# Autodesk Inventor assembly: Z Axis FR
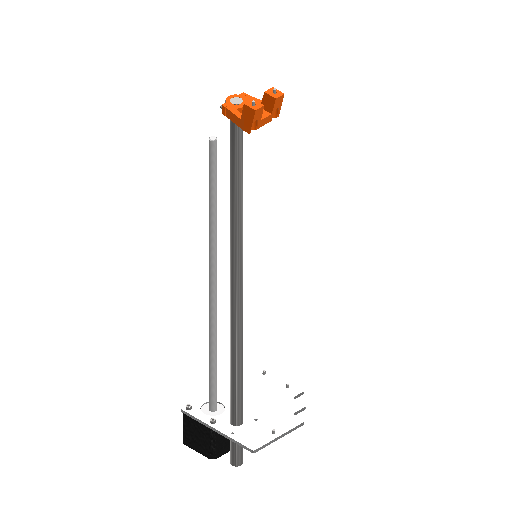
[picture p0: Inventor's stored thumbnail of the model, 512x512]
Saved by Autodesk Inventor 2023.2 (Build 272271000, 271)
## iProperties
Created: 2023-02-02
Part Number: Z Axis FR
Document SubType Name: Assembly
Designer: remop
Author: remop
## Documents named in this file (9)
- C:\Users\remop\OneDrive\Documents\Inventor\3D Printers\LuEVO\Mk5_FullKinematic\Z Axis Front Right.iam
- C:\Users\remop\OneDrive\Documents\Inventor\3D Printers\LuEVO\Mk5_FullKinematic\Z Axis Side Motor Mount.ipt
- C:\Users\remop\OneDrive\Documents\Inventor\3D Printers\LuEVO\Mk5_FullKinematic\Z Axis Motor.ipt
- C:\Users\remop\OneDrive\Documents\Inventor\3D Printers\LuEVO\Mk5_FullKinematic\Z Axis Guide.ipt
- C:\Users\remop\OneDrive\Documents\Inventor\3D Printers\LuEVO\Mk5_FullKinematic\Z Axis Top Brace.ipt
- C:\Users\remop\OneDrive\Documents\Inventor\Content Center Files\R2023\en-US\AS 1420\AS 1420 - 1973 - M3 x 6.ipt
- C:\Users\remop\OneDrive\Documents\Inventor\Content Center Files\R2023\en-US\AS 1420\AS 1420 - 1973 - M3 x 8.ipt
- C:\Users\remop\OneDrive\Documents\Inventor\3D Printers\LuEVO\Mk5_FullKinematic\Z Axis Top Brace Clamp.ipt
- C:\Users\remop\OneDrive\Documents\Inventor\Content Center Files\R2023\en-US\AS 1420\AS 1420 - 1973 - M3 x 12.ipt
## Components (16 placed, 8 different names)
1. Z Axis Side Motor Mount:1 — Rigid:1, Rigid:2, Angle:1, Insert:1, Insert:4, Insert:5, Insert:6, Insert:7, Insert:8, Insert:9
2. Z Axis Motor:1 — Rigid:1
3. Z Axis Guide:1 — Rigid:2, Mate:1, Flush:1
4. Z Axis Top Brace:1 — Mate:1, Flush:1, Angle:1, Insert:10, Insert:11, Flush:2
5. AS 1420 - Metric M3 x 6:1 — Insert:1
6. AS 1420 - Metric M3 x 6:4 — Insert:4
7. AS 1420 - Metric M3 x 6:5 — Insert:5
8. AS 1420 - Metric M3 x 6:6 — Insert:6
9. AS 1420 - Metric M3 x 6:7 — Insert:7
10. AS 1420 - Metric M3 x 6:8 — Insert:8
11. AS 1420 - Metric M3 x 6:9 — Insert:9
12. AS 1420 - Metric M3 x 8:1 — Insert:10
13. AS 1420 - Metric M3 x 8:2 — Insert:11
14. Z Axis Top Brace Clamp:1 — Flush:2, Insert:12, Rigid:3
15. AS 1420 - Metric M3 x 12:1 — Insert:12
16. AS 1420 - Metric M3 x 12:2 — Rigid:3
## Relationships (17: Insert 10, WeldJoint 3, Flush 2, Mate 1, Angle 1)
- Rigid:1 [WeldJoint]: Z Axis Side Motor Mount:1 ↔ Z Axis Motor:1
- Rigid:2 [WeldJoint] (42 mm): Z Axis Side Motor Mount:1 ↔ Z Axis Guide:1
- Mate:1: Z Axis Guide:1 ↔ Z Axis Top Brace:1
- Flush:1: Z Axis Guide:1 ↔ Z Axis Top Brace:1
- Angle:1 (0 deg): Z Axis Side Motor Mount:1 ↔ Z Axis Top Brace:1
- Insert:1: Z Axis Side Motor Mount:1 ↔ AS 1420 - Metric M3 x 6:1
- Insert:4: Z Axis Side Motor Mount:1 ↔ AS 1420 - Metric M3 x 6:4
- Insert:5: Z Axis Side Motor Mount:1 ↔ AS 1420 - Metric M3 x 6:5
- Insert:6: Z Axis Side Motor Mount:1 ↔ AS 1420 - Metric M3 x 6:6
- Insert:7: Z Axis Side Motor Mount:1 ↔ AS 1420 - Metric M3 x 6:7
- Insert:8: Z Axis Side Motor Mount:1 ↔ AS 1420 - Metric M3 x 6:8
- Insert:9: Z Axis Side Motor Mount:1 ↔ AS 1420 - Metric M3 x 6:9
- Insert:10: Z Axis Top Brace:1 ↔ AS 1420 - Metric M3 x 8:1
- Insert:11: Z Axis Top Brace:1 ↔ AS 1420 - Metric M3 x 8:2
- Flush:2: Z Axis Top Brace:1 ↔ Z Axis Top Brace Clamp:1
- Insert:12: Z Axis Top Brace Clamp:1 ↔ AS 1420 - Metric M3 x 12:1
- Rigid:3 [WeldJoint]: Z Axis Top Brace Clamp:1 ↔ AS 1420 - Metric M3 x 12:2
